# Autodesk Inventor assembly: Electrical Board Assembly
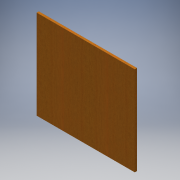
[picture p0: Inventor's stored thumbnail of the model, 180x180]
Saved by Autodesk Inventor 2016 (Build 200138000, 138)
## iProperties
Created: 2016-01-27
Part Number: Electrical Board Assembly
Document SubType Name: Assembly
Designer: PrashantBIA
Author: PrashantBIA
## Documents named in this file (5)
- C:\Users\PrashantBIA\Desktop\Robotics\Robot Assembly\Electronic Parts\Electrical Board Assembly.iam
- C:\Users\PrashantBIA\Desktop\Robotics\Robot Assembly\Electronic Parts\Electrical Board.ipt
- C:\Users\PrashantBIA\Desktop\Robotics\Robot Assembly\Electronic Parts\PDBoard.ipt
- C:\Users\PrashantBIA\Desktop\Robotics\Robot Assembly\Electronic Parts\Victor.ipt
- C:\Users\PrashantBIA\Desktop\Robotics\Robot Assembly\Electronic Parts\vrm.ipt
## Components (9 placed, 4 different names)
1. Electrical Board:1 — Mate:2, Angle:3, Mate:3, Mate:4, Mate:5, Mate:6, Mate:7, Mate:8, Mate:9, Angle:4, Angle:5, Angle:6, Angle:7, Angle:8, Angle:9, Angle:10
2. PDBoard:1 — Mate:2, Angle:3
3. Victor:1 — Mate:3, Angle:5
4. Victor:2 — Mate:4, Angle:8
5. Victor:3 — Mate:5, Angle:7
6. Victor:4 — Mate:8, Angle:6
7. Victor:5 — Mate:7, Angle:9
8. Victor:6 — Mate:6, Angle:10
9. vrm:1 — Mate:9, Angle:4
## Relationships (16: Mate 8, Angle 8)
- Mate:2: Electrical Board:1 ↔ PDBoard:1
- Angle:3 (0 deg): Electrical Board:1 ↔ PDBoard:1
- Mate:3: Electrical Board:1 ↔ Victor:1
- Mate:4: Electrical Board:1 ↔ Victor:2
- Mate:5: Electrical Board:1 ↔ Victor:3
- Mate:6: Electrical Board:1 ↔ Victor:6
- Mate:7: Electrical Board:1 ↔ Victor:5
- Mate:8: Electrical Board:1 ↔ Victor:4
- Mate:9: Electrical Board:1 ↔ vrm:1
- Angle:4 (0 deg): Electrical Board:1 ↔ vrm:1
- Angle:5 (0 deg): Electrical Board:1 ↔ Victor:1
- Angle:6 (0 deg): Electrical Board:1 ↔ Victor:4
- Angle:7 (0 deg): Electrical Board:1 ↔ Victor:3
- Angle:8 (0 deg): Electrical Board:1 ↔ Victor:2
- Angle:9 (0 deg): Electrical Board:1 ↔ Victor:5
- Angle:10 (0 deg): Electrical Board:1 ↔ Victor:6
